# Autodesk Inventor assembly: Turret ASM
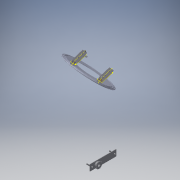
[picture p0: Inventor's stored thumbnail of the model, 180x180]
Saved by Autodesk Inventor 2017 (Build 210142000, 142)
## iProperties
Created: 2016-09-26
Part Number: Turret ASM
Document SubType Name: Assembly
Designer: Hanson
Author: Hanson
## Documents named in this file (12)
- \\Mac\Home\Desktop\bunnybots 2016\15102898-16-Bunnybot-CAD\Bunnybot-To_be_renamed\15102898-16-A-0000\15102898-16-A-0600\Turret ASM.iam
- \\Mac\Home\Desktop\bunnybots 2016\15102898-16-Bunnybot-CAD\Bunnybot-To_be_renamed\15102898-16-A-0000\15102898-16-A-0600\User Library-LazySusan 12inch.ipt
- \\Mac\Home\Desktop\bunnybots 2016\15102898-16-Bunnybot-CAD\Bunnybot-To_be_renamed\15102898-16-A-0000\15102898-16-A-0600\Large crossbeam.ipt
- \\Mac\Home\Desktop\bunnybots 2016\15102898-16-Bunnybot-CAD\Bunnybot-To_be_renamed\15102898-16-A-0000\15102898-16-A-0600\90480A195_LOW-STRENGTH STEEL HEX NUT.ipt
- \\Mac\Home\Desktop\bunnybots 2016\15102898-16-Bunnybot-CAD\Bunnybot-To_be_renamed\15102898-16-A-0000\15102898-16-A-0600\92196A277_18-8 STAINLESS STEEL SOCKET HEAD CAP SCREW.ipt
- \\Mac\Home\Desktop\bunnybots 2016\15102898-16-Bunnybot-CAD\Bunnybot-To_be_renamed\15102898-16-A-0000\15102898-16-A-0600\BAG motor top plate.ipt
- \\Mac\Home\Desktop\bunnybots 2016\15102898-16-Bunnybot-CAD\Bunnybot-To_be_renamed\15102898-16-A-0000\15102898-16-A-0600\92196A545_18-8 STAINLESS STEEL SOCKET HEAD CAP SCREW.ipt
- \\Mac\Home\Desktop\bunnybots 2016\15102898-16-Bunnybot-CAD\Bunnybot-To_be_renamed\15102898-16-A-0000\15102898-16-A-0600\plate mount nut.ipt
- \\Mac\Home\Desktop\bunnybots 2016\15102898-16-Bunnybot-CAD\Bunnybot-To_be_renamed\15102898-16-A-0000\15102898-16-A-0600\Main base bolt.ipt
- \\Mac\Home\Desktop\bunnybots 2016\15102898-16-Bunnybot-CAD\Bunnybot-To_be_renamed\15102898-16-A-0000\15102898-16-A-0600\lazy susan bushing.ipt
- \\Mac\Home\Desktop\bunnybots 2016\15102898-16-Bunnybot-CAD\Bunnybot-To_be_renamed\15102898-16-A-0000\15102898-16-A-0600\BAG motor\VersaPlanetary-1-Stage-with-BAG-Motor.iam
- \\Mac\Home\Desktop\bunnybots 2016\15102898-16-Bunnybot-CAD\Bunnybot-To_be_renamed\15102898-16-A-0000\15102898-16-A-0600\217-2642-STEP-20140807.ipt
## Components (24 placed, 11 different names)
1. User Library-LazySusan 12inch:1 — Mate:4, Mate:5, Mate:7, Mate:9, Mate:10, Mate:12, Mate:15
2. Large crossbeam:1 — Insert:16, Insert:17, Insert:18, Insert:21, Insert:22, Flush:1, Flush:2, Mate:17, Flush:3
3. Large crossbeam:2 — Insert:13, Insert:14, Insert:15, Insert:19, Insert:20, Insert:23, Insert:24, Flush:1, Mate:14, Flush:2, Mate:19
4. 92196A277_18-8 STAINLESS STEEL SOCKET HEAD CAP SCREW:1 — Insert:13
5. 92196A277_18-8 STAINLESS STEEL SOCKET HEAD CAP SCREW:2 — Insert:14
6. BAG motor top plate:1 — Insert:11, Insert:12, Mate:14, Flush:3, Mate:18, Flush:4
7. 92196A545_18-8 STAINLESS STEEL SOCKET HEAD CAP SCREW:1 — Insert:11
8. 92196A545_18-8 STAINLESS STEEL SOCKET HEAD CAP SCREW:2 — Insert:12, Mate:17
9. plate mount nut:1 — Insert:15
10. plate mount nut:2 — Insert:16
11. Main base bolt:1 — Insert:17, Mate:16
12. Main base bolt:2 — Insert:18, Mate:6, Mate:15
13. Main base bolt:3 — Insert:19, Mate:8
14. Main base bolt:4 — Insert:20, Mate:11
15. lazy susan bushing:1 — Insert:21, Mate:5
16. lazy susan bushing:2 — Insert:22
17. lazy susan bushing:3 — Insert:23
18. lazy susan bushing:4 — Insert:24, Mate:4
19. 90480A195_LOW-STRENGTH STEEL HEX NUT:1 — Mate:12, Mate:16
20. 90480A195_LOW-STRENGTH STEEL HEX NUT:2 — Mate:6, Mate:7
21. 90480A195_LOW-STRENGTH STEEL HEX NUT:3 — Mate:8, Mate:9
22. 90480A195_LOW-STRENGTH STEEL HEX NUT:4 — Mate:10, Mate:11
23. VersaPlanetary-1-Stage-with-BAG-Motor:1 [sub-assembly] — Mate:18, Mate:19, Flush:4, Mate:20, Mate:21, Flush:5
24. 217-2642-STEP-20140807:1 — Mate:20, Mate:21, Flush:5
## Relationships (36: Mate 17, Insert 14, Flush 5)
- Insert:11: BAG motor top plate:1 ↔ 92196A545_18-8 STAINLESS STEEL SOCKET HEAD CAP SCREW:1
- Insert:12: BAG motor top plate:1 ↔ 92196A545_18-8 STAINLESS STEEL SOCKET HEAD CAP SCREW:2
- Insert:13: Large crossbeam:2 ↔ 92196A277_18-8 STAINLESS STEEL SOCKET HEAD CAP SCREW:1
- Insert:14: Large crossbeam:2 ↔ 92196A277_18-8 STAINLESS STEEL SOCKET HEAD CAP SCREW:2
- Insert:15: Large crossbeam:2 ↔ plate mount nut:1
- Insert:16: Large crossbeam:1 ↔ plate mount nut:2
- Insert:17: Large crossbeam:1 ↔ Main base bolt:1
- Insert:18: Large crossbeam:1 ↔ Main base bolt:2
- Insert:19: Large crossbeam:2 ↔ Main base bolt:3
- Insert:20: Large crossbeam:2 ↔ Main base bolt:4
- Insert:21: Large crossbeam:1 ↔ lazy susan bushing:1
- Insert:22: Large crossbeam:1 ↔ lazy susan bushing:2
- Insert:23: Large crossbeam:2 ↔ lazy susan bushing:3
- Insert:24: Large crossbeam:2 ↔ lazy susan bushing:4
- Flush:1: Large crossbeam:1 ↔ Large crossbeam:2
- Mate:4: User Library-LazySusan 12inch:1 ↔ lazy susan bushing:4
- Mate:5: User Library-LazySusan 12inch:1 ↔ lazy susan bushing:1
- Mate:6: Main base bolt:2 ↔ 90480A195_LOW-STRENGTH STEEL HEX NUT:2
- Mate:7: User Library-LazySusan 12inch:1 ↔ 90480A195_LOW-STRENGTH STEEL HEX NUT:2
- Mate:8: Main base bolt:3 ↔ 90480A195_LOW-STRENGTH STEEL HEX NUT:3
- Mate:9: User Library-LazySusan 12inch:1 ↔ 90480A195_LOW-STRENGTH STEEL HEX NUT:3
- Mate:10: User Library-LazySusan 12inch:1 ↔ 90480A195_LOW-STRENGTH STEEL HEX NUT:4
- Mate:11: Main base bolt:4 ↔ 90480A195_LOW-STRENGTH STEEL HEX NUT:4
- Mate:12: User Library-LazySusan 12inch:1 ↔ 90480A195_LOW-STRENGTH STEEL HEX NUT:1
- Mate:14: Large crossbeam:2 ↔ BAG motor top plate:1
- Flush:2: Large crossbeam:1 ↔ Large crossbeam:2
- Mate:15: User Library-LazySusan 12inch:1 ↔ Main base bolt:2
- Mate:16: Main base bolt:1 ↔ 90480A195_LOW-STRENGTH STEEL HEX NUT:1
- Mate:17: Large crossbeam:1 ↔ 92196A545_18-8 STAINLESS STEEL SOCKET HEAD CAP SCREW:2
- Flush:3: Large crossbeam:1 ↔ BAG motor top plate:1
- Mate:18: BAG motor top plate:1 ↔ VersaPlanetary-1-Stage-with-BAG-Motor:1
- Mate:19: Large crossbeam:2 ↔ VersaPlanetary-1-Stage-with-BAG-Motor:1
- Flush:4: BAG motor top plate:1 ↔ VersaPlanetary-1-Stage-with-BAG-Motor:1
- Mate:20: VersaPlanetary-1-Stage-with-BAG-Motor:1 ↔ 217-2642-STEP-20140807:1
- Mate:21: VersaPlanetary-1-Stage-with-BAG-Motor:1 ↔ 217-2642-STEP-20140807:1
- Flush:5 (23.8125 mm): VersaPlanetary-1-Stage-with-BAG-Motor:1 ↔ 217-2642-STEP-20140807:1
